# Autodesk Inventor assembly: Assembly2
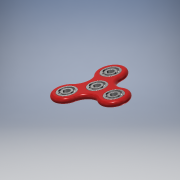
[picture p0: Inventor's stored thumbnail of the model, 180x180]
Saved by Autodesk Inventor 2018 (Build 220112000, 112)
## iProperties
Created: 2020-06-26
Part Number: Assembly2
Document SubType Name: Assembly
Designer: Brandon Portillo
Author: Brandon Portillo
## Documents named in this file (4)
- C:\Users\Brandon Portillo\Documents\Inventor\TO4\Assembly2.iam
- C:\Users\Brandon Portillo\Documents\Inventor\TO4\TO4.ipt
- C:\Users\Brandon Portillo\Documents\Inventor\TO4\Assembly2\Design Accelerator\Bearing1.iam
- C:\Users\Brandon Portillo\Documents\Inventor\TO4\Assembly2\Design Accelerator\Bearing2.iam
## Components (5 placed, 2 different names)
1. TO4:1 — Mate:1, Mate:2, Mate:3, Mate:4
2. Bearing:1 [sub-assembly] — Mate:1, Mate:2, Mate:5, Mate:6
3. Bearing:2 [sub-assembly] — Mate:3, Mate:4
4. Bearing:3 [sub-assembly]
5. Bearing:4 [sub-assembly]
## Component patterns: (3 elements, first: Bearing:2)
## Relationships (6: Mate 6)
- Mate:1: TO4:1 ↔ Bearing:1
- Mate:2: TO4:1 ↔ Bearing:1
- Mate:3: TO4:1 ↔ Bearing:2
- Mate:4: TO4:1 ↔ Bearing:2
- Mate:5: Bearing:1
- Mate:6: Bearing:1
